# Autodesk Inventor assembly: 00-00-Сборка
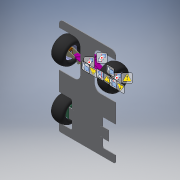
[picture p0: Inventor's stored thumbnail of the model, 180x180]
Saved by Autodesk Inventor 2018 (Build 220112000, 112)
## iProperties
Part Number: 00-00-Сборка
Material: Типовые
Document SubType Name: Assembly
Designer: sbnnl
Author: sbnnl
## Documents named in this file (8)
- D:\Загрузки\IMMO\00-00-Сборка.iam
- D:\Загрузки\IMMO\00-01-Платформа.ipt
- D:\Загрузки\IMMO\04-00-Привод передний.iam
- D:\Загрузки\IMMO\02-00-Двигатель.ipt
- D:\Загрузки\IMMO\05-01-Кронштейн верх.ipt
- D:\Загрузки\IMMO\05-01-Кронштейн низ.ipt
- D:\Загрузки\IMMO\01-00-Колесо.iam
- D:\Загрузки\IMMO\05-01-Кронштейн низ защита.ipt
## Components (7 placed, 7 different names)
1. 00-01-Платформа:1 — Совмещение:17, Совмещение:18, Совмещение:19, Совмещение:20, Совмещение:24, Заподлицо:1, Угол:1, С поворотом:1
2. 04-00-Привод передний:1 [sub-assembly] — Совмещение:18, Совмещение:19, Совмещение:20
3. 02-00-Двигатель:1 — Совмещение:21, Совмещение:22, Совмещение:25, Угол:1, Заподлицо:2, Заподлицо:3
4. 05-01-Кронштейн верх:1 — Совмещение:21, Совмещение:23, Заподлицо:3
5. 05-01-Кронштейн низ:1 — Совмещение:22, Совмещение:23, Совмещение:24
6. 01-00-Колесо:1 [sub-assembly] — Совмещение:25, Заподлицо:1, Заподлицо:2
7. 05-01-Кронштейн низ защита:1 — С поворотом:1
## Relationships (14: Mate 9, Flush 3, Angle 1, RevoluteJoint 1)
- Совмещение:17 [Mate]: 00-01-Платформа:1
- Совмещение:18 [Mate]: 00-01-Платформа:1 ↔ 04-00-Привод передний:1
- Совмещение:19 [Mate]: 00-01-Платформа:1 ↔ 04-00-Привод передний:1
- Совмещение:20 [Mate]: 00-01-Платформа:1 ↔ 04-00-Привод передний:1
- Совмещение:21 [Mate]: 02-00-Двигатель:1 ↔ 05-01-Кронштейн верх:1
- Совмещение:22 [Mate]: 02-00-Двигатель:1 ↔ 05-01-Кронштейн низ:1
- Совмещение:23 [Mate]: 05-01-Кронштейн верх:1 ↔ 05-01-Кронштейн низ:1
- Совмещение:24 [Mate]: 00-01-Платформа:1 ↔ 05-01-Кронштейн низ:1
- Совмещение:25 [Mate]: 02-00-Двигатель:1 ↔ 01-00-Колесо:1
- Заподлицо:1 [Flush] (14 mm): 00-01-Платформа:1 ↔ 01-00-Колесо:1
- Угол:1 [Angle] (0 deg): 00-01-Платформа:1 ↔ 02-00-Двигатель:1
- Заподлицо:2 [Flush] (30 mm): 02-00-Двигатель:1 ↔ 01-00-Колесо:1
- Заподлицо:3 [Flush]: 02-00-Двигатель:1 ↔ 05-01-Кронштейн верх:1
- С поворотом:1 [RevoluteJoint]: 00-01-Платформа:1 ↔ 05-01-Кронштейн низ защита:1
